# Autodesk Inventor assembly: 214
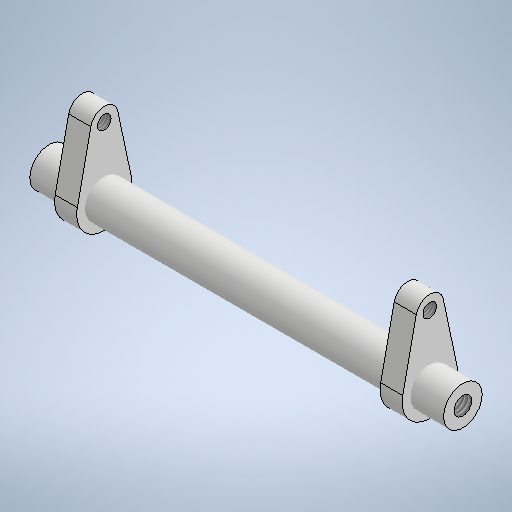
[picture p0: Inventor's stored thumbnail of the model, 512x512]
Saved by Autodesk Inventor 2025 (Build 290162010, 162A)
## iProperties
Created: 2024-06-09
Part Number: 214
Document SubType Name: Assembly
Designer: Fabri
Author: Fabri
## Documents named in this file (3)
- C:\Users\Fabri\Documents\Inventor\Paddle\214.iam
- C:\Users\Fabri\Documents\Inventor\Paddle\214.1.ipt
- C:\Users\Fabri\Documents\Inventor\Paddle\214.3.ipt
## Components (3 placed, 2 different names)
1. 214.1:1 — Insert:1
2. 214.1:2 — Insert:2
3. 214.3:1 — Insert:1, Insert:2
## Relationships (2: Insert 2)
- Insert:1 (-10 mm): 214.1:1 ↔ 214.3:1
- Insert:2 (-10 mm): 214.1:2 ↔ 214.3:1
